# Autodesk Inventor assembly: selection system
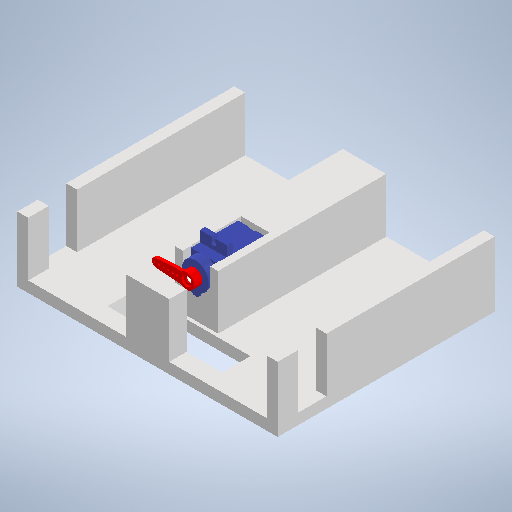
[picture p0: Inventor's stored thumbnail of the model, 512x512]
Saved by Autodesk Inventor 2025.3 (Build 293356000, 356)
## iProperties
Created: 2026-04-13
Part Number: selection system
Document SubType Name: Assembly
Designer: kamal
Author: kamal
## Documents named in this file (5)
- C:\Users\kamal\OneDrive\Desktop\Personal\semester 4\Basics of Mechatronics\Full Assembly\selection system.iam
- C:\Users\kamal\OneDrive\Desktop\Personal\semester 4\Basics of Mechatronics\Full Assembly\Selection Body V1.ipt
- C:\Users\kamal\OneDrive\Desktop\Personal\semester 4\Basics of Mechatronics\Full Assembly\SG90_Model_A.ipt
- C:\Users\kamal\OneDrive\Desktop\Personal\semester 4\Basics of Mechatronics\Full Assembly\SG90_Arm_Original.ipt
- C:\Users\kamal\OneDrive\Desktop\Personal\semester 4\Basics of Mechatronics\Mechanisms\Sorting tool\Sorting tool\Servo_Shaft_select_V1.ipt
## Components (4 placed, 4 different names)
1. Selection Body V1:1 — Mate:1, Mate:2, Mate:3
2. SG90_Model_A:1 — Mate:1, Mate:2, Mate:3, Insert:1
3. SG90_Arm_Original:1 — Insert:1, Mate:4, Insert:2
4. Servo_Shaft_select_V1:1 — Mate:4, Insert:2
## Relationships (6: Mate 4, Insert 2)
- Mate:1: Selection Body V1:1 ↔ SG90_Model_A:1
- Mate:2: Selection Body V1:1 ↔ SG90_Model_A:1
- Mate:3: Selection Body V1:1 ↔ SG90_Model_A:1
- Insert:1: SG90_Model_A:1 ↔ SG90_Arm_Original:1
- Mate:4: SG90_Arm_Original:1 ↔ Servo_Shaft_select_V1:1
- Insert:2: SG90_Arm_Original:1 ↔ Servo_Shaft_select_V1:1
